# Autodesk Inventor assembly: Chassis Assembly
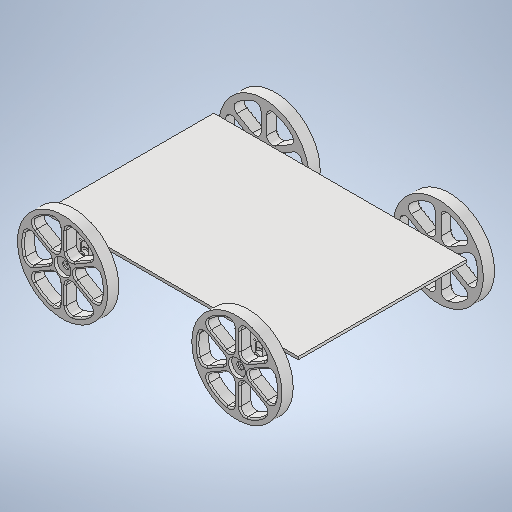
[picture p0: Inventor's stored thumbnail of the model, 512x512]
Saved by Autodesk Inventor 2025.2 (Build 292293000, 293)
## iProperties
Created: 2025-01-16
Part Number: Chassis Assembly
Document SubType Name: Assembly
Designer: Matt Tidd
Author: Matt Tidd
## Documents named in this file (5)
- C:\Users\mtidd2\Desktop\H2A\CAD\Chassis_Design\Chassis Assembly.iam
- C:\Users\mtidd2\Desktop\H2A\CAD\Motors_and_Wheels\520 DC Gear Motor Bracket Assembly.iam
- C:\Users\mtidd2\Desktop\H2A\CAD\Chassis_Design\ChassisTest.ipt
- C:\Users\mtidd2\Desktop\H2A\CAD\Motors_and_Wheels\520 DC Gear Motor Wheel Coupler.ipt
- C:\Users\mtidd2\Desktop\H2A\CAD\Motors_and_Wheels\PLA Wheel Frame.ipt
## Components (13 placed, 4 different names)
1. ChassisTest:1 — Mate:1, Mate:2, Mate:3, Mate:4, Mate:5, Mate:6, Mate:7, Mate:8
2. 520 DC Gear Motor Bracket Assembly:1 [sub-assembly] — Mate:1, Mate:2, Mate:10
3. 520 DC Gear Motor Bracket Assembly:2 [sub-assembly] — Mate:3, Mate:4, Mate:9
4. 520 DC Gear Motor Bracket Assembly:3 [sub-assembly] — Mate:7, Mate:8, Mate:11
5. 520 DC Gear Motor Bracket Assembly:4 [sub-assembly] — Mate:5, Mate:6, Mate:12
6. 520 DC Gear Motor Wheel Coupler:1 — Mate:9, Mate:17, Mate:18
7. 520 DC Gear Motor Wheel Coupler:2 — Mate:10, Mate:19, Mate:20
8. 520 DC Gear Motor Wheel Coupler:3 — Mate:11, Mate:15, Mate:16
9. 520 DC Gear Motor Wheel Coupler:4 — Mate:12, Mate:13, Mate:14
10. PLA Wheel Frame:1 — Mate:15, Mate:16
11. PLA Wheel Frame:2 — Mate:13, Mate:14
12. PLA Wheel Frame:3 — Mate:19, Mate:20
13. PLA Wheel Frame:4 — Mate:17, Mate:18
## Relationships (20: Mate 20)
- Mate:1: ChassisTest:1 ↔ 520 DC Gear Motor Bracket Assembly:1
- Mate:2 (50 mm): ChassisTest:1 ↔ 520 DC Gear Motor Bracket Assembly:1
- Mate:3: ChassisTest:1 ↔ 520 DC Gear Motor Bracket Assembly:2
- Mate:4 (50 mm): ChassisTest:1 ↔ 520 DC Gear Motor Bracket Assembly:2
- Mate:5 (50 mm): ChassisTest:1 ↔ 520 DC Gear Motor Bracket Assembly:4
- Mate:6: ChassisTest:1 ↔ 520 DC Gear Motor Bracket Assembly:4
- Mate:7: ChassisTest:1 ↔ 520 DC Gear Motor Bracket Assembly:3
- Mate:8 (50 mm): ChassisTest:1 ↔ 520 DC Gear Motor Bracket Assembly:3
- Mate:9: 520 DC Gear Motor Bracket Assembly:2 ↔ 520 DC Gear Motor Wheel Coupler:1
- Mate:10: 520 DC Gear Motor Bracket Assembly:1 ↔ 520 DC Gear Motor Wheel Coupler:2
- Mate:11: 520 DC Gear Motor Bracket Assembly:3 ↔ 520 DC Gear Motor Wheel Coupler:3
- Mate:12: 520 DC Gear Motor Bracket Assembly:4 ↔ 520 DC Gear Motor Wheel Coupler:4
- Mate:13: 520 DC Gear Motor Wheel Coupler:4 ↔ PLA Wheel Frame:2
- Mate:14: 520 DC Gear Motor Wheel Coupler:4 ↔ PLA Wheel Frame:2
- Mate:15: 520 DC Gear Motor Wheel Coupler:3 ↔ PLA Wheel Frame:1
- Mate:16: 520 DC Gear Motor Wheel Coupler:3 ↔ PLA Wheel Frame:1
- Mate:17: 520 DC Gear Motor Wheel Coupler:1 ↔ PLA Wheel Frame:4
- Mate:18: 520 DC Gear Motor Wheel Coupler:1 ↔ PLA Wheel Frame:4
- Mate:19: 520 DC Gear Motor Wheel Coupler:2 ↔ PLA Wheel Frame:3
- Mate:20: 520 DC Gear Motor Wheel Coupler:2 ↔ PLA Wheel Frame:3
